# Autodesk Inventor assembly: Zed_Assembly
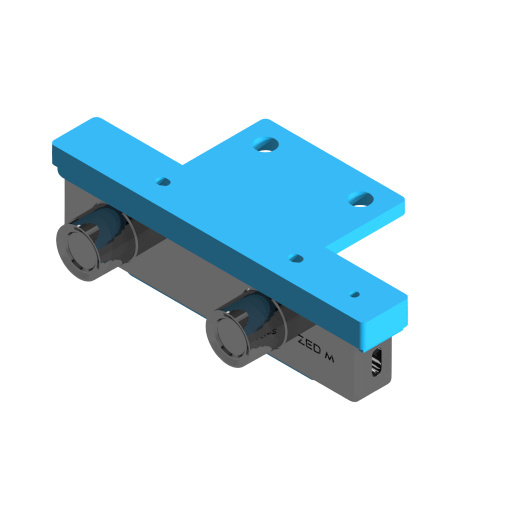
[picture p0: Inventor's stored thumbnail of the model, 512x512]
Saved by Autodesk Inventor 2023.1 (Build 271208000, 208)
## iProperties
Created: 2022-09-25
Part Number: Zed_Assembly
Document SubType Name: Assembly
Designer: Jakob
Author: Jakob
## Documents named in this file (3)
- C:\Users\Jakob\OneDrive\thesis\zedMount\Zed_Assembly.iam
- C:\Users\Jakob\OneDrive\thesis\zedMount\ZED_Mini_Holder_v5.ipt
- C:\Users\Jakob\OneDrive\thesis\zedMount\ZEDM.ipt
## Components (2 placed, 2 different names)
1. ZED_Mini_Holder_v5:1 — Mate:1
2. ZEDM:1 — Mate:1
## Relationships (1: Mate 1)
- Mate:1: ZED_Mini_Holder_v5:1 ↔ ZEDM:1
